# Autodesk Inventor assembly: Tensioner4b1_MIR
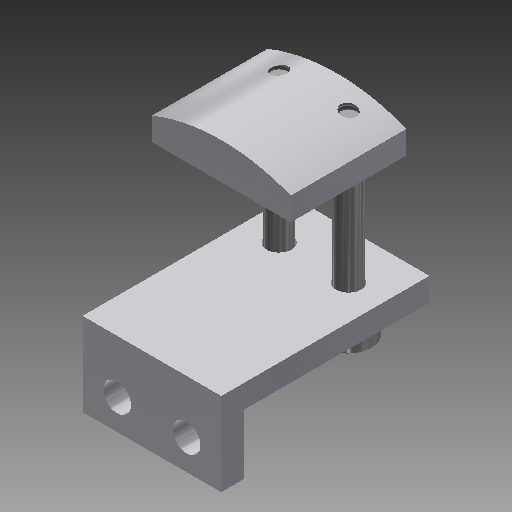
[picture p0: Inventor's stored thumbnail of the model, 512x512]
Saved by Autodesk Inventor 2017 (Build 210142000, 142)
## iProperties
Created: 2018-05-19
Part Number: Tensioner4b1_MIR
Document SubType Name: Assembly
Designer: User
Author: User
## Documents named in this file (4)
- C:\Robotics\CAD\2018-19_CAD\Offseason\Tensioner4b1_MIR.iam
- C:\Robotics\CAD\2018-19_CAD\Offseason\TensionerPlate4b1_MIR.ipt
- C:\Robotics\CAD\2018-19_CAD\Offseason\TensionerPusher41_MIR.ipt
- C:\Robotics\CAD\COTSParts\Fasteners\92012A506_.125D.75L_ALLOY STEEL PRECISION SHOULDER SCREW1_MIR.ipt
## Components (4 placed, 3 different names)
1. TensionerPlate4b1_MIR:1 — Mate:3, Mate:2, Mate:1
2. TensionerPusher41_MIR:1 — Mate:3, Insert:1, Insert:2
3. 92012A506_.125D.75L_ALLOY STEEL PRECISION SHOULDER SCREW1_MIR:1 — Mate:2, Insert:1
4. 92012A506_.125D.75L_ALLOY STEEL PRECISION SHOULDER SCREW1_MIR:2 — Mate:1, Insert:2
## Relationships (5: Mate 3, Insert 2)
- Mate:3: TensionerPlate4b1_MIR:1 ↔ TensionerPusher41_MIR:1
- Mate:2: TensionerPlate4b1_MIR:1 ↔ 92012A506_.125D.75L_ALLOY STEEL PRECISION SHOULDER SCREW1_MIR:1
- Insert:1: TensionerPusher41_MIR:1 ↔ 92012A506_.125D.75L_ALLOY STEEL PRECISION SHOULDER SCREW1_MIR:1
- Mate:1: TensionerPlate4b1_MIR:1 ↔ 92012A506_.125D.75L_ALLOY STEEL PRECISION SHOULDER SCREW1_MIR:2
- Insert:2: TensionerPusher41_MIR:1 ↔ 92012A506_.125D.75L_ALLOY STEEL PRECISION SHOULDER SCREW1_MIR:2
